# Autodesk Inventor assembly: BrakeLight
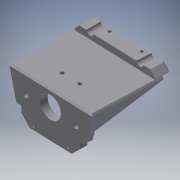
[picture p0: Inventor's stored thumbnail of the model, 180x180]
Saved by Autodesk Inventor 2019 (Build 230136000, 136)
## iProperties
Created: 2019-08-14
Part Number: BrakeLight
Document SubType Name: Assembly
Designer: steve
Author: steve
## Documents named in this file (4)
- C:\Users\steve\Documents\GitHub\Motorcycle\CAD Files\BrakeLight.iam
- C:\Users\steve\Documents\GitHub\Motorcycle\CAD Files\Brake_Light_Base_Plate.ipt
- C:\Users\steve\Documents\GitHub\Motorcycle\CAD Files\Bar_Mount_Bottom.ipt
- C:\Users\steve\Documents\GitHub\Motorcycle\CAD Files\License_plate_mount.ipt
## Components (3 placed, 3 different names)
1. Bar_Mount_Bottom:1 — Rigid:1
2. Brake_Light_Base_Plate:1 — Rigid:1, Rigid:2
3. License_plate_mount:1 — Rigid:2
## Relationships (2: WeldJoint 2)
- Rigid:1 [WeldJoint]: Bar_Mount_Bottom:1 ↔ Brake_Light_Base_Plate:1
- Rigid:2 [WeldJoint]: Brake_Light_Base_Plate:1 ↔ License_plate_mount:1
